# Autodesk Inventor assembly: Plow_Assembly
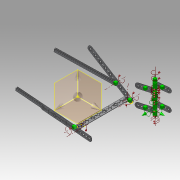
[picture p0: Inventor's stored thumbnail of the model, 180x180]
Saved by Autodesk Inventor 2016 (Build 200138000, 138)
## iProperties
Created: 2015-10-23
Part Number: Plow_Assembly
Document SubType Name: Assembly
Designer: Delta
Author: Delta
## Documents named in this file (10)
- C:\Robotics\CAD\2015-16\custom cad parts\Plow_Assembly.iam
- C:\Robotics\CAD\2015-16\COTSParts\Tetrix\Tetrix bracket - angle.ipt
- C:\Robotics\CAD\2015-16\COTSParts\Actobotics\585 parts\585398.ipt
- C:\Robotics\CAD\2015-16\custom cad parts\Tetrix Max Flat 288mm.ipt
- C:\Robotics\CAD\2015-16\COTSParts\Tetrix\Tetrix shaft 100mm.ipt
- C:\Robotics\CAD\2015-16\COTSParts\Tetrix\Bronze bushing.ipt
- C:\Robotics\CAD\2015-16\COTSParts\Tetrix\Tetrix Lego Adapter.ipt
- C:\Robotics\CAD\2015-16\COTSParts\Tetrix\Tetrix shaft collar.ipt
- C:\Robotics\CAD\2015-16\COTSParts\Tetrix\Tetrix Hub - axle_MIR.ipt
- C:\Robotics\CAD\2015-16\COTSParts\Tetrix\Pitsco Education-739273.ipt
## Components (29 placed, 9 different names)
1. Tetrix bracket - angle:1 — Insert:1, Mate:6, Mate:8, Angle:1
2. Tetrix bracket - angle:2 — Insert:30, Mate:7, Mate:9
3. 585398:1 — Insert:8
4. 585398:2 — Insert:4
5. Tetrix Max Flat 288mm:1 — Insert:4, Insert:30
6. Tetrix Max Flat 288mm:2 — Insert:1, Insert:8
7. Tetrix Max Flat 288mm:3 — Mate:6, Mate:7, Mate:8, Mate:9, Angle:1
8. Tetrix shaft 100mm:1
9. Bronze bushing:1
10. Bronze bushing:2
11. Bronze bushing:3
12. Bronze bushing:4
13. Bronze bushing:5
14. Tetrix shaft 100mm:2
15. Tetrix Lego Adapter:1
16. Tetrix Lego Adapter:2
17. Tetrix Lego Adapter:3
18. Tetrix shaft collar:1
19. Tetrix Hub - axle_MIR:1
20. Tetrix Hub - axle_MIR:2
21. Bronze bushing:6
22. Tetrix Lego Adapter:4
23. Tetrix shaft collar:2
24. Bronze bushing:7
25. Bronze bushing:8
26. Pitsco Education-739273:1
27. Pitsco Education-739273:2
28. Pitsco Education-739273:3
29. Pitsco Education-739273:4
## Relationships (35: Insert 25, Mate 9, Angle 1)
- Insert:1: Tetrix bracket - angle:1 ↔ Tetrix Max Flat 288mm:2
- Insert:4: 585398:2 ↔ Tetrix Max Flat 288mm:1
- Insert:8: 585398:1 ↔ Tetrix Max Flat 288mm:2
- [Insert]: Tetrix shaft 100mm:1 ↔ Tetrix Hub - axle_MIR:1
- [Insert]: Tetrix shaft 100mm:2 ↔ Tetrix Hub - axle_MIR:2
- [Mate]: Tetrix shaft 100mm:1 ↔ Bronze bushing:4
- [Mate]: Bronze bushing:4 ↔ Tetrix Hub - axle_MIR:1
- [Insert] (2.032 mm): Tetrix Hub - axle_MIR:1 ↔ Tetrix Hub - axle_MIR:2
- [Insert]: Bronze bushing:1 ↔ Tetrix Hub - axle_MIR:2
- [Insert]: Bronze bushing:1 ↔ Tetrix Lego Adapter:2
- [Insert]: Bronze bushing:3 ↔ Tetrix Lego Adapter:2
- [Insert]: Bronze bushing:3 ↔ Bronze bushing:5
- [Insert]: Bronze bushing:5 ↔ Tetrix Lego Adapter:1
- [Insert]: Bronze bushing:2 ↔ Tetrix Lego Adapter:1
- [Insert]: Bronze bushing:2 ↔ Tetrix shaft collar:1
- [Insert]: Bronze bushing:4 ↔ Tetrix Lego Adapter:3
- [Insert]: Tetrix Lego Adapter:3 ↔ Bronze bushing:7
- [Insert]: Bronze bushing:6 ↔ Bronze bushing:7
- [Insert]: Bronze bushing:6 ↔ Tetrix Lego Adapter:4
- [Insert]: Tetrix Lego Adapter:4 ↔ Bronze bushing:8
- [Insert]: Tetrix shaft collar:2 ↔ Bronze bushing:8
- [Insert]: Tetrix Lego Adapter:4 ↔ Pitsco Education-739273:1
- [Insert]: Tetrix Lego Adapter:4 ↔ Pitsco Education-739273:1
- [Insert]: Tetrix Lego Adapter:2 ↔ Pitsco Education-739273:2
- [Mate]: Tetrix Lego Adapter:2 ↔ Pitsco Education-739273:2
- [Insert]: Tetrix Lego Adapter:3 ↔ Pitsco Education-739273:4
- [Mate]: Tetrix Lego Adapter:3 ↔ Pitsco Education-739273:4
- [Insert]: Tetrix Lego Adapter:1 ↔ Pitsco Education-739273:3
- [Mate]: Tetrix Lego Adapter:1 ↔ Pitsco Education-739273:3
- Insert:30: Tetrix bracket - angle:2 ↔ Tetrix Max Flat 288mm:1
- Mate:6: Tetrix bracket - angle:1 ↔ Tetrix Max Flat 288mm:3
- Mate:7: Tetrix bracket - angle:2 ↔ Tetrix Max Flat 288mm:3
- Mate:8: Tetrix bracket - angle:1 ↔ Tetrix Max Flat 288mm:3
- Mate:9: Tetrix bracket - angle:2 ↔ Tetrix Max Flat 288mm:3
- Angle:1 (0 deg): Tetrix bracket - angle:1 ↔ Tetrix Max Flat 288mm:3
## Named parameters: d19_d0 = 0 mm, d22_d28 = 0 mm, d23_d29 = 0 mm, d24_d30 = 0 mm, d27_d6 = 0 mm, d32_d11 = 0 mm, d33_d12 = 0 mm, d35_d14 = 0 mm
